# Autodesk Inventor assembly: Drive Arm
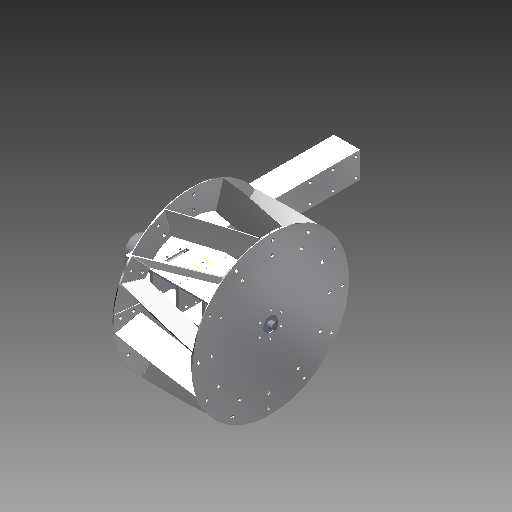
[picture p0: Inventor's stored thumbnail of the model, 512x512]
Saved by Autodesk Inventor 2019 (Build 230136000, 136)
## iProperties
Created: 2018-10-12
Part Number: Drive Arm
Document SubType Name: Assembly
Designer: Adhik
Mass: 2954.71 g
Surface Area: 9053.91 cm^2
Volume: 1103.34 cm^3
Density: 2.67797 g/cm^3
Author: Adhik
## Documents named in this file (13)
- E:\CAD\Julie\Drive Arm.iam
- E:\CAD\Julie\Arm 18 inch.ipt
- E:\CAD\Julie\Gearbox.iam
- E:\CAD\Julie\Arm 2 inch A.ipt
- E:\CAD\Julie\Arm 2 inch B.ipt
- E:\CAD\Julie\Arm 2 inch C.ipt
- E:\CAD\Julie\3775.ipt
- E:\CAD\Julie\Arm Bearing.ipt
- E:\CAD\Julie\Shaft.ipt
- E:\CAD\Julie\Wheel.iam
- E:\CAD\Julie\Shaft Coupler.ipt
- E:\CAD\Julie\Gearbox Shaft.ipt
- E:\CAD\Julie\Gearbox.ipt
## Components (13 placed, 11 different names)
1. Arm 18 inch:1 — Mate:1, Flush:1, Flush:2, Mate:3, Mate:16
2. Gearbox:1 [sub-assembly] — Mate:1, Mate:6, Mate:7, Mate:8, Mate:9, Mate:11
3. Arm 2 inch A:1 — Flush:1, Flush:2, Mate:3, Mate:4, Flush:4, Flush:5, Mate:6, Mate:7, Mate:17, Mate:18, Mate:19
4. Arm 2 inch B:1 — Mate:4, Mate:5, Flush:3, Flush:4, Flush:5, Flush:6
5. Arm 2 inch C:1 — Mate:5, Flush:3, Flush:6, Insert:1, Insert:2
6. 3775:1 — Mate:8, Mate:9, Mate:16, Mate:20
7. Arm Bearing:1 — Insert:2, Mate:10, Mate:13
8. Arm Bearing:2 — Insert:1, Mate:15
9. Shaft:1 — Mate:10, Mate:11, Mate:12, Mate:14
10. Wheel:1 [sub-assembly] — Mate:12, Mate:13
11. Shaft Coupler:1 — Mate:14, Mate:15
12. Gearbox Shaft:1 — Insert:3
13. Gearbox:2 — Insert:3, Mate:17, Mate:18, Mate:19, Mate:20
## Relationships (28: Mate 19, Flush 6, Insert 3)
- Mate:1: Arm 18 inch:1 ↔ Gearbox:1
- Flush:1: Arm 18 inch:1 ↔ Arm 2 inch A:1
- Flush:2: Arm 18 inch:1 ↔ Arm 2 inch A:1
- Mate:3: Arm 18 inch:1 ↔ Arm 2 inch A:1
- Mate:4: Arm 2 inch A:1 ↔ Arm 2 inch B:1
- Mate:5: Arm 2 inch B:1 ↔ Arm 2 inch C:1
- Flush:3: Arm 2 inch B:1 ↔ Arm 2 inch C:1
- Flush:4: Arm 2 inch A:1 ↔ Arm 2 inch B:1
- Flush:5: Arm 2 inch A:1 ↔ Arm 2 inch B:1
- Flush:6: Arm 2 inch B:1 ↔ Arm 2 inch C:1
- Mate:6: Gearbox:1 ↔ Arm 2 inch A:1
- Mate:7: Gearbox:1 ↔ Arm 2 inch A:1
- Mate:8: Gearbox:1 ↔ 3775:1
- Mate:9: Gearbox:1 ↔ 3775:1
- Insert:1: Arm 2 inch C:1 ↔ Arm Bearing:2
- Insert:2: Arm 2 inch C:1 ↔ Arm Bearing:1
- Mate:10: Arm Bearing:1 ↔ Shaft:1
- Mate:11: Gearbox:1 ↔ Shaft:1
- Mate:12: Shaft:1 ↔ Wheel:1
- Mate:13: Arm Bearing:1 ↔ Wheel:1
- Mate:14: Shaft:1 ↔ Shaft Coupler:1
- Mate:15: Arm Bearing:2 ↔ Shaft Coupler:1
- Mate:16: Arm 18 inch:1 ↔ 3775:1
- Insert:3: Gearbox Shaft:1 ↔ Gearbox:2
- Mate:17: Arm 2 inch A:1 ↔ Gearbox:2
- Mate:18: Arm 2 inch A:1 ↔ Gearbox:2
- Mate:19: Arm 2 inch A:1 ↔ Gearbox:2
- Mate:20: 3775:1 ↔ Gearbox:2
